# Autodesk Inventor assembly: MainAssembly2
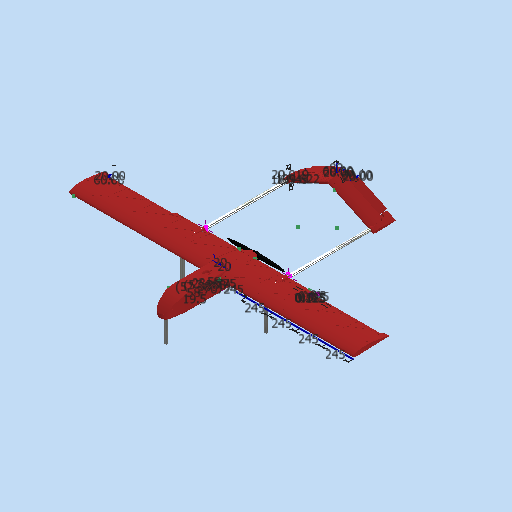
[picture p0: Inventor's stored thumbnail of the model, 512x512]
Saved by Autodesk Inventor 2027 (Build 310192060, 192F)
## iProperties
Created: 2026-04-16
Part Number: MainAssembly2
Document SubType Name: Assembly
Designer: mateo
Author: mateo
## Documents named in this file (22)
- C:\GitHub\SWIFT-UAV\System_development\Pelican\structural_model\v0.3.0\MainAssembly\MainAssembly2.iam
- C:\GitHub\SWIFT-UAV\System_development\Pelican\structural_model\v0.3.0\Parts\Fuselage\Fueselage.ipt
- C:\GitHub\SWIFT-UAV\System_development\Pelican\structural_model\v0.3.0\Parts\Wings\WingBox.ipt
- C:\GitHub\SWIFT-UAV\System_development\Pelican\structural_model\v0.3.0\Parts\Cover\FrontCover.ipt
- C:\GitHub\SWIFT-UAV\System_development\Pelican\structural_model\v0.3.0\Parts\Aluminum_20x20\20x20x1295ExtrudedAluminum.ipt
- C:\GitHub\SWIFT-UAV\System_development\Pelican\structural_model\v0.3.0\Parts\Aluminum_20x20\20x20x1295ExtrudedAluminum_MIR.ipt
- C:\GitHub\SWIFT-UAV\System_development\Pelican\structural_model\v0.3.0\Parts\Wings\WingLeft_v0.1.ipt
- C:\GitHub\SWIFT-UAV\System_development\Pelican\structural_model\v0.3.0\Parts\Wings\WingLeft_v0.1_MIR.ipt
- C:\GitHub\SWIFT-UAV\System_development\Pelican\structural_model\v0.3.0\Parts\Aluminum_20x20\20x20x800ExtrudedAluminum.ipt
- C:\GitHub\SWIFT-UAV\System_development\Pelican\structural_model\v0.3.0\Parts\Aluminum_20x20\20x20x800ExtrudedAluminum_MIR.ipt
- C:\GitHub\SWIFT-UAV\System_development\Pelican\structural_model\v0.3.0\Parts\Tail\Tail_V0.0.ipt
- C:\GitHub\SWIFT-UAV\System_development\Pelican\structural_model\v0.3.0\Parts\Tail\Vtail_V0.0.ipt
- C:\GitHub\SWIFT-UAV\System_development\Pelican\structural_model\v0.3.0\Parts\Tail\Vtail_MIR_V0.0.ipt
- C:\GitHub\SWIFT-UAV\System_development\Pelican\structural_model\v0.3.0\Parts\Wings\AlerionLeft_V0.1.ipt
- C:\GitHub\SWIFT-UAV\System_development\Pelican\structural_model\v0.3.0\Parts\Wings\AlerionLeft_MIR_V0.1.ipt
- C:\GitHub\SWIFT-UAV\System_development\Pelican\structural_model\v0.3.0\Avionics\X7215\X7215\X7215.ipt
- C:\GitHub\SWIFT-UAV\System_development\Pelican\structural_model\v0.3.0\Parts\Accessorys\Prop.ipt
- C:\GitHub\SWIFT-UAV\System_development\Pelican\structural_model\v0.3.0\Parts\Aluminum_20x20\20x20x785ExtrudedAluminum.ipt
- C:\GitHub\SWIFT-UAV\System_development\Pelican\structural_model\v0.3.0\Parts\Aluminum_20x20\20x20x230ExtrudedAluminum.ipt
- C:\GitHub\SWIFT-UAV\System_development\Pelican\structural_model\v0.3.0\Parts\Aluminum_20x20\20x20x330ExtrudedAluminum.ipt
- C:\Users\sunsh\OneDrive\Documents\GitHub\SWIFT-UAV\System_development\Pelican\structural_model\v0.3.0\Parts\4in_Wheel.ipt
- C:\GitHub\SWIFT-UAV\System_development\Pelican\structural_model\v0.3.0\Parts\Accessorys\UAV_Stand.ipt
## Components (27 placed, 21 different names)
1. Fueselage:1 — Mate:1, Mate:2, Mate:3, Mate:4, Flush:1, Mate:5, Mate:6, Mate:7, Insert:5, Mate:24, Mate:26, Mate:27
2. WingBox:1 — Mate:3, Mate:4, Flush:1, Mate:8, Mate:9, Flush:2, Mate:13, Mate:14
3. FrontCover:1 — Mate:5, Mate:6, Mate:7
4. 20x20x1295ExtrudedAluminum:1 — Mate:9, Flush:2, Mate:10, Mate:12, Mate:18, Mate:29
5. 20x20x1295ExtrudedAluminum_MIR:1 — Mate:8, Mate:10, Mate:11, Mate:17
6. WingLeft_v0.1:1 — Mate:11, Mate:13, Mate:15, Insert:3
7. WingLeft_v0.1_MIR:1 — Mate:12, Mate:14, Mate:16, Insert:4
8. 20x20x800ExtrudedAluminum:1 — Mate:15, Mate:17, Mate:20, Mate:21, Mate:22
9. 20x20x800ExtrudedAluminum_MIR:1 — Mate:16, Mate:18, Mate:23
10. Tail_V0.0:1 — Mate:20, Mate:21, Mate:22, Mate:23, Insert:1, Insert:2
11. Vtail_V0.0:1 — Insert:2
12. Vtail_MIR_V0.0:1 — Insert:1
13. AlerionLeft_V0.1:1 — Insert:4
14. AlerionLeft_MIR_V0.1:1 — Insert:3
15. X7215:1 — Insert:5, Insert:6
16. Prop:1 — Insert:6
17. 20x20x785ExtrudedAluminum:1 — Mate:24, Mate:26, Mate:27, Mate:28, Mate:37
18. 20x20x230ExtrudedAluminum:1 — Mate:28, Mate:33, Mate:34
19. 20x20x330ExtrudedAluminum:1 — Mate:29, Mate:31, Mate:32
20. 20x20x330ExtrudedAluminum:2 — Mate:35, Mate:36
21. 4in_Wheel:1 — Mate:34
22. 4in_Wheel:2 — Mate:33
23. 4in_Wheel:3 — Mate:31
24. 4in_Wheel:4 — Mate:32
25. 4in_Wheel:5 — Mate:36
26. 4in_Wheel:6 — Mate:35
27. UAV_Stand:1 — Mate:37
## Relationships (42: Mate 34, Insert 6, Flush 2)
- Mate:1: Fueselage:1
- Mate:2: Fueselage:1
- Mate:3: Fueselage:1 ↔ WingBox:1
- Mate:4: Fueselage:1 ↔ WingBox:1
- Flush:1: Fueselage:1 ↔ WingBox:1
- Mate:5: Fueselage:1 ↔ FrontCover:1
- Mate:6: Fueselage:1 ↔ FrontCover:1
- Mate:7: Fueselage:1 ↔ FrontCover:1
- Mate:8: WingBox:1 ↔ 20x20x1295ExtrudedAluminum_MIR:1
- Mate:9: WingBox:1 ↔ 20x20x1295ExtrudedAluminum:1
- Flush:2: WingBox:1 ↔ 20x20x1295ExtrudedAluminum:1
- Mate:10: 20x20x1295ExtrudedAluminum:1 ↔ 20x20x1295ExtrudedAluminum_MIR:1
- Mate:11: 20x20x1295ExtrudedAluminum_MIR:1 ↔ WingLeft_v0.1:1
- Mate:12: 20x20x1295ExtrudedAluminum:1 ↔ WingLeft_v0.1_MIR:1
- Mate:13: WingBox:1 ↔ WingLeft_v0.1:1
- Mate:14: WingBox:1 ↔ WingLeft_v0.1_MIR:1
- Mate:15: WingLeft_v0.1:1 ↔ 20x20x800ExtrudedAluminum:1
- Mate:16: WingLeft_v0.1_MIR:1 ↔ 20x20x800ExtrudedAluminum_MIR:1
- Mate:17: 20x20x1295ExtrudedAluminum_MIR:1 ↔ 20x20x800ExtrudedAluminum:1
- Mate:18: 20x20x1295ExtrudedAluminum:1 ↔ 20x20x800ExtrudedAluminum_MIR:1
- Mate:20 (76.2 mm): 20x20x800ExtrudedAluminum:1 ↔ Tail_V0.0:1
- Mate:21: 20x20x800ExtrudedAluminum:1 ↔ Tail_V0.0:1
- Mate:22: 20x20x800ExtrudedAluminum:1 ↔ Tail_V0.0:1
- Mate:23: 20x20x800ExtrudedAluminum_MIR:1 ↔ Tail_V0.0:1
- Insert:1: Tail_V0.0:1 ↔ Vtail_MIR_V0.0:1
- Insert:2: Tail_V0.0:1 ↔ Vtail_V0.0:1
- Insert:3 (5 mm): WingLeft_v0.1:1 ↔ AlerionLeft_MIR_V0.1:1
- Insert:4 (5 mm): WingLeft_v0.1_MIR:1 ↔ AlerionLeft_V0.1:1
- Insert:5 (-12.7 mm): Fueselage:1 ↔ X7215:1
- Insert:6 (-5.08 mm): X7215:1 ↔ Prop:1
- Mate:24: Fueselage:1 ↔ 20x20x785ExtrudedAluminum:1
- Mate:26: Fueselage:1 ↔ 20x20x785ExtrudedAluminum:1
- Mate:27: Fueselage:1 ↔ 20x20x785ExtrudedAluminum:1
- Mate:28: 20x20x785ExtrudedAluminum:1 ↔ 20x20x230ExtrudedAluminum:1
- Mate:29: 20x20x1295ExtrudedAluminum:1 ↔ 20x20x330ExtrudedAluminum:1
- Mate:31: 20x20x330ExtrudedAluminum:1 ↔ 4in_Wheel:3
- Mate:32: 20x20x330ExtrudedAluminum:1 ↔ 4in_Wheel:4
- Mate:33: 20x20x230ExtrudedAluminum:1 ↔ 4in_Wheel:2
- Mate:34: 20x20x230ExtrudedAluminum:1 ↔ 4in_Wheel:1
- Mate:35: 20x20x330ExtrudedAluminum:2 ↔ 4in_Wheel:6
- Mate:36: 20x20x330ExtrudedAluminum:2 ↔ 4in_Wheel:5
- Mate:37: 20x20x785ExtrudedAluminum:1 ↔ UAV_Stand:1
